# Autodesk Inventor assembly: PitchGears
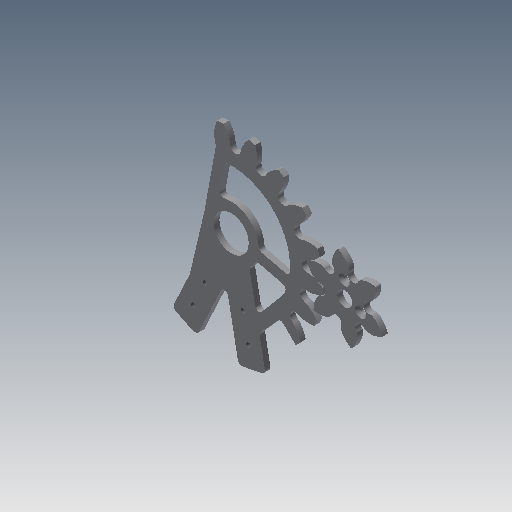
[picture p0: Inventor's stored thumbnail of the model, 512x512]
Saved by Autodesk Inventor 2019.4 (Build 234330000, 330)
## iProperties
Created: 2019-06-11
Part Number: PitchGears
Document SubType Name: Assembly
Designer: AzLIer
Mass: 12.5954 g
Surface Area: 112.764 cm^2
Volume: 12.5954 cm^3
Density: 1 g/cm^3
Author: AzLIer
## Documents named in this file (3)
- E:\ロボ研\キャチロボ\キャチロボ2019\アーム2019\PitchGears\PitchGears.iam
- E:\ロボ研\キャチロボ\キャチロボ2019\アーム2019\PitchGears\m5-18.ipt
- E:\ロボ研\キャチロボ\キャチロボ2019\アーム2019\PitchGears\m5-6(dis0.4).ipt
## Components (2 placed, 2 different names)
1. m5-18:1 — メイト:1, メイト:2, Fit, 回転:1, フラッシュ:1
2. m5-6(dis0.4):1 — メイト:1, メイト:3, Fit, 回転:1, Drive, フラッシュ:1
## Relationships (7: Mate 4, RelateRotation 1, Angle 1, Flush 1)
- メイト:1 [Mate] (61.8122 mm): m5-18:1 ↔ m5-6(dis0.4):1
- メイト:2 [Mate]: m5-18:1
- メイト:3 [Mate]: m5-6(dis0.4):1
- Fit [Mate]: m5-18:1 ↔ m5-6(dis0.4):1
- 回転:1 [RelateRotation] (3 ul): m5-18:1 ↔ m5-6(dis0.4):1
- Drive [Angle] (30 deg): m5-6(dis0.4):1
- フラッシュ:1 [Flush]: m5-18:1 ↔ m5-6(dis0.4):1
